# Autodesk Inventor assembly: Camera Assembly with new Cap
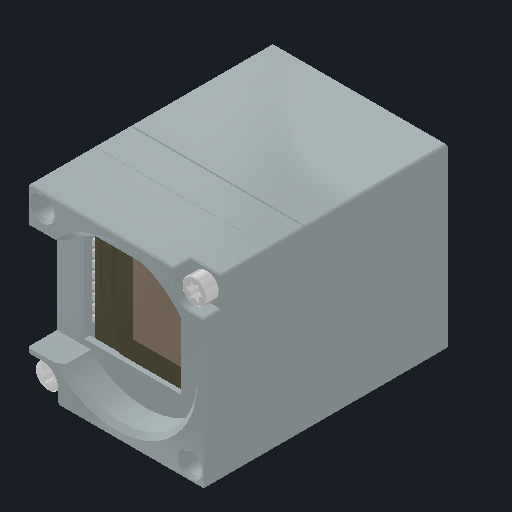
[picture p0: Inventor's stored thumbnail of the model, 512x512]
Saved by Autodesk Inventor 2026 (Build 300175000, 175)
## iProperties
Created: 2026-03-18
Part Number: Camera Assembly with new Cap
Document SubType Name: Assembly
Designer: FiolkaLab
Author: FiolkaLab
## Documents named in this file (3)
- E:\Muaaz\Baseplate\Detection\Camera\Camera Assembly with new Cap.iam
- E:\Muaaz\Baseplate\Detection\Camera\MU196xR-ON-ADPT-MU-CX3-TC-V_01-STP-DWL_3dmodel\MU196xR-ON-ADPT-MU-CX3-TC-V_01-STP-DWL_3dmodel\MU196xR-ON-ADPT-MU-CX3-TC-V_01-STP-DWL_3dmodel.ipt
- E:\Muaaz\Baseplate\Detection\Camera\Camera Edit for Cap for Machining.iam
## Components (2 placed, 2 different names)
1. MU196xR-ON-ADPT-MU-CX3-TC-V_01-STP-DWL_3dmodel:1 — Flush:1, Mate:1, Mate:2
2. Camera Edit for Cap for Machining:1 [sub-assembly] — Flush:1, Mate:1, Mate:2
## Relationships (3: Mate 2, Flush 1)
- Flush:1: MU196xR-ON-ADPT-MU-CX3-TC-V_01-STP-DWL_3dmodel:1 ↔ Camera Edit for Cap for Machining:1
- Mate:1: MU196xR-ON-ADPT-MU-CX3-TC-V_01-STP-DWL_3dmodel:1 ↔ Camera Edit for Cap for Machining:1
- Mate:2: MU196xR-ON-ADPT-MU-CX3-TC-V_01-STP-DWL_3dmodel:1 ↔ Camera Edit for Cap for Machining:1
